# Autodesk Inventor assembly: folivora
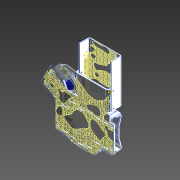
[picture p0: Inventor's stored thumbnail of the model, 180x180]
Saved by Autodesk Inventor 2018 (Build 220112000, 112)
## iProperties
Created: 2018-05-16
Part Number: folivora
Material: 一般
Document SubType Name: Assembly
Designer: NaMACHAN
Mass: 288.127 g
Surface Area: 1001.27 cm^2
Volume: 118.04 cm^3
Density: 2.44093 g/cm^3
Author: NaMACHAN
## Documents named in this file (21)
- C:\Users\NaMACHAN\Dropbox\Project\original\folivora\inventor\folivora.iam
- C:\Users\NaMACHAN\Dropbox\Project\original\folivora\inventor\Part6.ipt
- C:\Users\NaMACHAN\Dropbox\Project\original\folivora\inventor\baseframe.ipt
- C:\Users\NaMACHAN\Dropbox\Project\original\folivora\inventor\keyplate3.ipt
- C:\Users\NaMACHAN\Dropbox\Project\original\folivora\inventor\keyplate4.ipt
- C:\Users\NaMACHAN\Dropbox\Project\original\folivora\inventor\keyL.ipt
- C:\Users\NaMACHAN\Dropbox\Project\original\folivora\inventor\ball.ipt
- C:\Users\NaMACHAN\Dropbox\Project\original\folivora\inventor\trackball-base.ipt
- C:\Users\NaMACHAN\Dropbox\Project\original\folivora\inventor\trackball-shaft.ipt
- C:\Users\NaMACHAN\Dropbox\Project\original\folivora\inventor\bearing.ipt
- C:\Users\NaMACHAN\Dropbox\Project\original\folivora\inventor\bearingcover.ipt
- C:\Users\NaMACHAN\Dropbox\Project\original\folivora\inventor\trackball_l.ipt
- C:\Users\NaMACHAN\Dropbox\Project\original\folivora\inventor\trackball-cover.ipt
- C:\Users\NaMACHAN\Dropbox\Project\original\folivora\inventor\trackball-spacer.ipt
- C:\Users\NaMACHAN\Dropbox\Project\original\folivora\inventor\palmrest.ipt
- C:\Users\NaMACHAN\Dropbox\Project\original\folivora\inventor\folivora\AIP\FEA\cjjue1qww.fins
- C:\Users\NaMACHAN\Dropbox\Project\original\folivora\inventor\folivora\AIP\FEA\cjjue1qww.fsat
- C:\Users\NaMACHAN\Dropbox\Project\original\folivora\inventor\folivora\AIP\FEA\cjjue1qww.ftes
- C:\Users\NaMACHAN\Dropbox\Project\original\folivora\inventor\folivora\AIP\FEA\cjjue1qww.fwiz
- C:\Users\NaMACHAN\Dropbox\Project\original\folivora\inventor\folivora\AIP\FEA\cjjue1r1c.fmsh
- C:\Users\NaMACHAN\Dropbox\Project\original\folivora\inventor\folivora\AIP\FEA\cjjue1r1d.fres
## Components (38 placed, 14 different names)
1. Part6:1
2. baseframe:1 — メイト:31, メイト:32, メイト:33, メイト:34, メイト:37, メイト:38, メイト:39, メイト:40, メイト:43, メイト:79, メイト:80, メイト:89, メイト:94, メイト:114, メイト:137, メイト:138, メイト:139
3. keyL:1 — メイト:1, メイト:2, メイト:3, 角度:1, メイト:33
4. keyplate4:1 — メイト:1, メイト:2, メイト:3, メイト:4, メイト:5, 角度:1, メイト:46, メイト:95
5. keyL:2 — メイト:4, メイト:5, メイト:37, メイト:43, フラッシュ:5, フラッシュ:12, フラッシュ:14
6. keyplate3:1 — メイト:6, メイト:7, メイト:8, メイト:9, メイト:10, 角度:2, メイト:44, メイト:45
7. keyL:3 — メイト:7, メイト:10, 角度:2, メイト:32
8. keyL:4 — メイト:6, メイト:8, メイト:9, メイト:40, フラッシュ:3, フラッシュ:4
9. keyplate3:2 — メイト:44
10. keyL:5 — メイト:31
11. keyL:6 — メイト:39, フラッシュ:3
12. keyL:7 — メイト:34
13. keyplate4:2 — メイト:45, メイト:46
14. keyL:8 — メイト:38, フラッシュ:4, フラッシュ:5
15. ball:1 — メイト:105, メイト:115
16. trackball-base:1 — メイト:52, メイト:53, メイト:54, メイト:55, メイト:56, メイト:57, メイト:58, メイト:59, メイト:60, メイト:61, メイト:62, メイト:63, フラッシュ:15, メイト:105, フラッシュ:16, メイト:117, メイト:118, メイト:119, メイト:120, メイト:124, メイト:125
17. trackball-shaft:1 — メイト:49, メイト:52, メイト:53, メイト:54
18. bearing:1 — メイト:49, メイト:55
19. trackball-shaft:2 — メイト:56, メイト:57, メイト:59
20. bearing:2 — メイト:58
21. trackball-shaft:3 — メイト:60, メイト:61, メイト:62
22. bearing:3 — メイト:63
23. bearingcover:1 — フラッシュ:15, フラッシュ:16, メイト:115, メイト:121, メイト:122, メイト:123, メイト:124, メイト:125, メイト:134, メイト:135, メイト:136
24. keyplate3:3
25. keyL:11 — メイト:80
26. keyL:12 — メイト:79, フラッシュ:13
27. keyL:14 — メイト:89, フラッシュ:12, フラッシュ:13, メイト:93
28. keyL:15 — メイト:94
29. keyplate4:3 — メイト:93, フラッシュ:14, メイト:95
30. trackball_l:1 — メイト:114, メイト:121, メイト:122, メイト:123
31. trackball-shaft:4 — メイト:116, メイト:117, メイト:118, メイト:119
32. bearing:4 — メイト:116, メイト:120
33. trackball-cover:1 — メイト:126, メイト:127, メイト:128, メイト:129, メイト:130, メイト:131, メイト:132, メイト:133
34. trackball-spacer:1 — メイト:126, メイト:130, メイト:136
35. trackball-spacer:2 — メイト:129, メイト:131, メイト:135
36. trackball-spacer:3 — メイト:128, メイト:133
37. trackball-spacer:4 — メイト:127, メイト:132, メイト:134
38. palmrest:1 — メイト:137, メイト:138, メイト:139
## Relationships (102: Mate 88, Flush 8, Angle 6)
- メイト:1 [Mate]: keyL:1 ↔ keyplate4:1
- メイト:2 [Mate] (1.5 mm): keyL:1 ↔ keyplate4:1
- メイト:3 [Mate] (15 mm): keyL:1 ↔ keyplate4:1
- メイト:4 [Mate]: keyplate4:1 ↔ keyL:2
- メイト:5 [Mate] (1.5 mm): keyplate4:1 ↔ keyL:2
- メイト:6 [Mate] (1.5 mm): keyplate3:1 ↔ keyL:4
- メイト:7 [Mate]: keyplate3:1 ↔ keyL:3
- メイト:8 [Mate]: keyplate3:1 ↔ keyL:4
- メイト:9 [Mate] (10 mm): keyplate3:1 ↔ keyL:4
- メイト:10 [Mate] (1.5 mm): keyplate3:1 ↔ keyL:3
- 角度:1 [Angle] (0 deg): keyL:1 ↔ keyplate4:1
- 角度:2 [Angle] (0 deg): keyplate3:1 ↔ keyL:3
- [Mate] (1.5 mm): keyplate3:2 ↔ keyL:6
- [Mate]: keyplate3:2 ↔ keyL:5
- [Mate]: keyplate3:2 ↔ keyL:6
- [Mate] (10 mm): keyplate3:2 ↔ keyL:6
- [Mate] (1.5 mm): keyplate3:2 ↔ keyL:5
- [Angle] (0 deg): keyplate3:2 ↔ keyL:5
- [Mate]: keyL:7 ↔ keyplate4:2
- [Mate] (1.5 mm): keyL:7 ↔ keyplate4:2
- [Mate] (15 mm): keyL:7 ↔ keyplate4:2
- [Mate]: keyplate4:2 ↔ keyL:8
- [Mate] (1.5 mm): keyplate4:2 ↔ keyL:8
- [Angle] (0 deg): keyL:7 ↔ keyplate4:2
- メイト:31 [Mate]: baseframe:1 ↔ keyL:5
- メイト:32 [Mate]: baseframe:1 ↔ keyL:3
- メイト:33 [Mate]: baseframe:1 ↔ keyL:1
- メイト:34 [Mate]: baseframe:1 ↔ keyL:7
- メイト:37 [Mate]: baseframe:1 ↔ keyL:2
- メイト:38 [Mate]: baseframe:1 ↔ keyL:8
- メイト:39 [Mate]: baseframe:1 ↔ keyL:6
- メイト:40 [Mate]: baseframe:1 ↔ keyL:4
- メイト:43 [Mate]: baseframe:1 ↔ keyL:2
- フラッシュ:3 [Flush]: keyL:4 ↔ keyL:6
- メイト:44 [Mate]: keyplate3:1 ↔ keyplate3:2
- メイト:45 [Mate]: keyplate3:1 ↔ keyplate4:2
- メイト:46 [Mate]: keyplate4:1 ↔ keyplate4:2
- フラッシュ:4 [Flush] (18 mm): keyL:4 ↔ keyL:8
- フラッシュ:5 [Flush] (3 mm): keyL:2 ↔ keyL:8
- メイト:49 [Mate]: trackball-shaft:1 ↔ bearing:1
- [Mate]: trackball-shaft:2 ↔ bearing:2
- [Mate]: trackball-shaft:3 ↔ bearing:3
- メイト:52 [Mate] (1.5 mm): trackball-base:1 ↔ trackball-shaft:1
- メイト:53 [Mate] (1.5 mm): trackball-base:1 ↔ trackball-shaft:1
- メイト:54 [Mate]: trackball-base:1 ↔ trackball-shaft:1
- メイト:55 [Mate] (0.5 mm): trackball-base:1 ↔ bearing:1
- メイト:56 [Mate] (1.5 mm): trackball-base:1 ↔ trackball-shaft:2
- メイト:57 [Mate] (1.5 mm): trackball-base:1 ↔ trackball-shaft:2
- メイト:58 [Mate] (0.5 mm): trackball-base:1 ↔ bearing:2
- メイト:59 [Mate]: trackball-base:1 ↔ trackball-shaft:2
- メイト:60 [Mate] (1.5 mm): trackball-base:1 ↔ trackball-shaft:3
- メイト:61 [Mate] (1.5 mm): trackball-base:1 ↔ trackball-shaft:3
- メイト:62 [Mate]: trackball-base:1 ↔ trackball-shaft:3
- メイト:63 [Mate] (0.5 mm): trackball-base:1 ↔ bearing:3
- [Mate] (1.5 mm): keyplate3:3 ↔ keyL:12
- [Mate]: keyplate3:3 ↔ keyL:11
- [Mate]: keyplate3:3 ↔ keyL:12
- [Mate] (10 mm): keyplate3:3 ↔ keyL:12
- [Mate] (1.5 mm): keyplate3:3 ↔ keyL:11
- [Angle] (0 deg): keyplate3:3 ↔ keyL:11
- メイト:79 [Mate]: baseframe:1 ↔ keyL:12
- メイト:80 [Mate]: baseframe:1 ↔ keyL:11
- メイト:89 [Mate]: baseframe:1 ↔ keyL:14
- フラッシュ:12 [Flush] (-3 mm): keyL:2 ↔ keyL:14
- フラッシュ:13 [Flush] (3 mm): keyL:12 ↔ keyL:14
- [Mate]: keyL:15 ↔ keyplate4:3
- [Mate] (1.5 mm): keyL:15 ↔ keyplate4:3
- [Mate] (15 mm): keyL:15 ↔ keyplate4:3
- [Angle] (0 deg): keyL:15 ↔ keyplate4:3
- メイト:93 [Mate] (1.5 mm): keyL:14 ↔ keyplate4:3
- メイト:94 [Mate]: baseframe:1 ↔ keyL:15
- フラッシュ:14 [Flush] (3 mm): keyL:2 ↔ keyplate4:3
- メイト:95 [Mate]: keyplate4:1 ↔ keyplate4:3
- フラッシュ:15 [Flush]: trackball-base:1 ↔ bearingcover:1
- メイト:105 [Mate]: ball:1 ↔ trackball-base:1
- メイト:114 [Mate]: baseframe:1 ↔ trackball_l:1
- フラッシュ:16 [Flush]: trackball-base:1 ↔ bearingcover:1
- メイト:115 [Mate] (6.4 mm): ball:1 ↔ bearingcover:1
- メイト:116 [Mate]: trackball-shaft:4 ↔ bearing:4
- メイト:117 [Mate] (1.5 mm): trackball-base:1 ↔ trackball-shaft:4
- メイト:118 [Mate] (1.5 mm): trackball-base:1 ↔ trackball-shaft:4
- メイト:119 [Mate]: trackball-base:1 ↔ trackball-shaft:4
- メイト:120 [Mate] (0.5 mm): trackball-base:1 ↔ bearing:4
- メイト:121 [Mate]: bearingcover:1 ↔ trackball_l:1
- メイト:122 [Mate]: bearingcover:1 ↔ trackball_l:1
- メイト:123 [Mate]: bearingcover:1 ↔ trackball_l:1
- メイト:124 [Mate]: trackball-base:1 ↔ bearingcover:1
- メイト:125 [Mate]: trackball-base:1 ↔ bearingcover:1
- メイト:126 [Mate]: trackball-cover:1 ↔ trackball-spacer:1
- メイト:127 [Mate]: trackball-cover:1 ↔ trackball-spacer:4
- メイト:128 [Mate]: trackball-cover:1 ↔ trackball-spacer:3
- メイト:129 [Mate]: trackball-cover:1 ↔ trackball-spacer:2
- メイト:130 [Mate]: trackball-cover:1 ↔ trackball-spacer:1
- メイト:131 [Mate]: trackball-cover:1 ↔ trackball-spacer:2
- メイト:132 [Mate]: trackball-cover:1 ↔ trackball-spacer:4
- メイト:133 [Mate]: trackball-cover:1 ↔ trackball-spacer:3
- メイト:134 [Mate]: bearingcover:1 ↔ trackball-spacer:4
- メイト:135 [Mate]: bearingcover:1 ↔ trackball-spacer:2
- メイト:136 [Mate]: bearingcover:1 ↔ trackball-spacer:1
- メイト:137 [Mate]: baseframe:1 ↔ palmrest:1
- メイト:138 [Mate]: baseframe:1 ↔ palmrest:1
- メイト:139 [Mate]: baseframe:1 ↔ palmrest:1
## Named parameters: sa_0 = 7.4e-12, sa_1 = -5000, sa_2 = 4e-13, sa_3 = -1.32e-11, sa_4 = -5000, sa_5 = -4.2e-12, sa_6 = -2.8e-12, sa_7 = -5000, sa_8 = -2.3e-12, sa_9 = -1e-12, sa_10 = -5000, sa_11 = -3.7e-12, sa_12 = 2.78e-11, sa_13 = -5000, sa_14 = 7e-12, sa_15 = 1.85e-11, sa_16 = -5000, sa_17 = 3.9e-12, d377_d369 = 1.5 mm, d378_d370 = 0 mm, d379_d371 = 0 mm, d380_d372 = 10 mm, d381_d373 = 1.5 mm, d382_d375 = 0 deg, d383_d366 = 1.5 mm, d385_d374 = 0 deg, d386_d362 = 0 mm, d387_d363 = 1.5 mm, d388_d364 = 15 mm, d389_d365 = 0 mm, d430_d429 = 0 mm, d431_d429 = 0 mm, d459_d377_d369 = 1.5 mm, d460_d378_d370 = 0 mm, d461_d379_d371 = 0 mm, d462_d380_d372 = 10 mm, d463_d381_d373 = 1.5 mm, d464_d382_d375 = 0 deg, d487_d362 = 0 mm, d488_d363 = 1.5 mm, d489_d364 = 15 mm, d490_d374 = 0 deg
note: some values were not read from the file. Shown as the stored number, unit unknown: "sa_0", "sa_1", "sa_2", "sa_3", "sa_4", "sa_5", "sa_6", "sa_7", "sa_8", "sa_9", "sa_10", "sa_11", "sa_12", "sa_13", "sa_14", "sa_15", "sa_16", "sa_17".
